# Autodesk Inventor assembly: FilterWheel-Dynamixel(MX28)
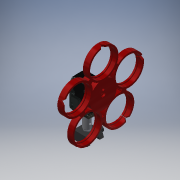
[picture p0: Inventor's stored thumbnail of the model, 180x180]
Saved by Autodesk Inventor 2017 (Build 210142000, 142)
## iProperties
Created: 2022-04-15
Part Number: FilterWheel-Dynamixel(MX28)
Document SubType Name: Assembly
Designer: Nikita
Author: Nikita
## Documents named in this file (6)
- C:\Users\Nikita\Documents\Nikita-UZH\mesoSPIM\CAD\FilterWheel-2inch\FilterWheel-Dynamixel(MX28).iam
- C:\Users\Nikita\Documents\Nikita-UZH\mesoSPIM\CAD\FilterWheel-2inch\MX-28AT_AR.ipt
- C:\Users\Nikita\Documents\Nikita-UZH\mesoSPIM\CAD\FilterWheel-2inch\FR07-S101.ipt
- C:\Users\Nikita\Documents\Nikita-UZH\mesoSPIM\CAD\FilterWheel-2inch\FilterWheel-2inch-5pos.ipt
- D:\mesoSPIM-Fabian\CAD_files\mesoSPIM_design_benchtop_V2\library\Thorlabs\posts\12_7_mm_posts\TR30.ipt
- C:\Users\Nikita\Documents\Nikita-UZH\mesoSPIM\CAD\Library\Thorlabs\Rail\RC1.ipt
## Components (5 placed, 5 different names)
1. MX-28AT_AR:1 — Mate:1, Insert:1, Angle:1, Insert:2
2. FR07-S101:1 — Mate:1, Insert:1, Angle:1, Insert:3
3. FilterWheel-2inch-5pos:1 — Insert:2, Angle:2
4. TR30:1 — Insert:3, Insert:4
5. RC1:1 — Insert:4, Angle:2
## Relationships (7: Insert 4, Angle 2, Mate 1)
- Mate:1: MX-28AT_AR:1 ↔ FR07-S101:1
- Insert:1: MX-28AT_AR:1 ↔ FR07-S101:1
- Angle:1 (0 deg): MX-28AT_AR:1 ↔ FR07-S101:1
- Insert:2: MX-28AT_AR:1 ↔ FilterWheel-2inch-5pos:1
- Insert:3: FR07-S101:1 ↔ TR30:1
- Insert:4: TR30:1 ↔ RC1:1
- Angle:2 (0 deg): FilterWheel-2inch-5pos:1 ↔ RC1:1
